# Autodesk Inventor assembly: board_box_bottom_with_holders
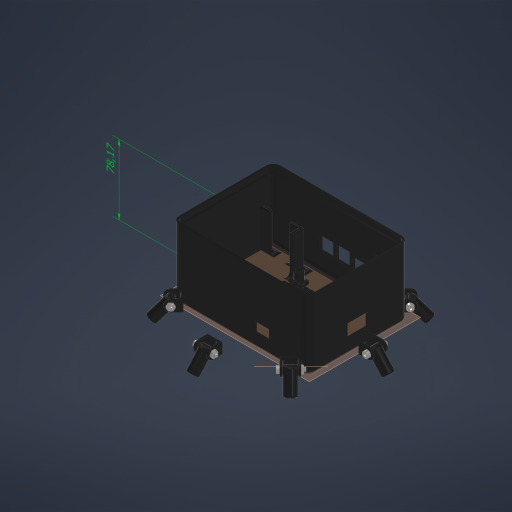
[picture p0: Inventor's stored thumbnail of the model, 512x512]
Saved by Autodesk Inventor 2023 (Build 270158030, 158C)
## iProperties
Created: 2022-07-17
Part Number: board_box_bottom_with_holders
Document SubType Name: Assembly
Designer: Norbert Ligas
Author: Norbert Ligas
## Documents named in this file (3)
- C:\Users\norbe\Repozytoria\NormalMapScanner\3D_modeling\construction\parts\board_box\board_box_bottom_with_holders.iam
- C:\Users\norbe\Repozytoria\NormalMapScanner\3D_modeling\construction\parts\board_box\board_box_bottom.ipt
- C:\Users\norbe\Repozytoria\NormalMapScanner\3D_modeling\construction\parts\board_box\board_box_bar_holder.iam
## Components (9 placed, 2 different names)
1. board_box_bottom:1 — Mate:1, Angle:1, Angle:2, Angle:3, Mate:3, Angle:4
2. board_box_bar_holder:1 [sub-assembly] — Mate:4, Flush:1
3. board_box_bar_holder:2 [sub-assembly]
4. board_box_bar_holder:3 [sub-assembly]
5. board_box_bar_holder:4 [sub-assembly] — Mate:5
6. board_box_bar_holder:5 [sub-assembly]
7. board_box_bar_holder:6 [sub-assembly]
8. board_box_bar_holder:7 [sub-assembly]
9. board_box_bar_holder:8 [sub-assembly]
## Component patterns: (8 elements, first: board_box_bar_holder:1)
## Relationships (10: Mate 5, Angle 4, Flush 1)
- Mate:1: board_box_bottom:1
- Mate:2
- Angle:1 (0 deg): board_box_bottom:1
- Angle:2 (0 deg): board_box_bottom:1
- Angle:3 (0 deg): board_box_bottom:1
- Mate:3: board_box_bottom:1
- Angle:4 (0 deg): board_box_bottom:1
- Mate:4: board_box_bar_holder:1
- Flush:1: board_box_bar_holder:1
- Mate:5: board_box_bar_holder:4
